# Autodesk Inventor assembly: Ensamble v2
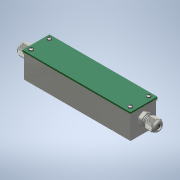
[picture p0: Inventor's stored thumbnail of the model, 180x180]
Saved by Autodesk Inventor 2021 (Build 250183000, 183)
## iProperties
Created: 2021-03-08
Part Number: Ensamble v2
Material: Generic
Document SubType Name: Assembly
Designer: Usuario
Author: Usuario
## Documents named in this file (8)
- C:\Users\Usuario\Desktop\INVENTOR\v 0.2\Ensamble v2.iam
- C:\Users\Usuario\Desktop\INVENTOR\v 0.2\base inferior.ipt
- C:\Users\Usuario\Desktop\INVENTOR\Componentes\PG7 Cable Gland.ipt
- C:\Users\Usuario\Desktop\INVENTOR\v 0.2\tapa.ipt
- C:\Users\Usuario\Desktop\INVENTOR\Componentes\Arduino\Arduino Nano R3 ATmega 328P.iam
- C:\Users\Usuario\Desktop\INVENTOR\Componentes\rs485.ipt
- C:\Users\Usuario\Desktop\INVENTOR\Componentes\SX1308_STEPUP_DCDC.ipt
- C:\Users\Usuario\Documents\Inventor\Content Center Files\R2021\en-US\BS EN ISO 7045 H\EN ISO 7045 - M3 x 10 - 4.8 - H(1).ipt
## Components (11 placed, 7 different names)
1. base inferior:1 — Insert:1, Insert:2, Mate:1, Flush:1, Mate:2, Mate:3, Mate:4
2. PG7 Cable Gland:1 — Insert:1
3. PG7 Cable Gland:2 — Insert:2
4. tapa:1 — Mate:1, Flush:1, Insert:3, Insert:4, Insert:5, Insert:6
5. Arduino Nano R3 ATmega 328P:1 [sub-assembly] — Mate:3
6. rs485:1 — Mate:4
7. SX1308_STEPUP_DCDC:1 — Mate:2
8. BS EN ISO 7045 H - Metric M3 x 10 - 4.8 - H:1 — Insert:4
9. BS EN ISO 7045 H - Metric M3 x 10 - 4.8 - H:2 — Insert:3
10. BS EN ISO 7045 H - Metric M3 x 10 - 4.8 - H:3 — Insert:6
11. BS EN ISO 7045 H - Metric M3 x 10 - 4.8 - H:4 — Insert:5
## Relationships (11: Insert 6, Mate 4, Flush 1)
- Insert:1: base inferior:1 ↔ PG7 Cable Gland:1
- Insert:2: base inferior:1 ↔ PG7 Cable Gland:2
- Mate:1: base inferior:1 ↔ tapa:1
- Flush:1: base inferior:1 ↔ tapa:1
- Mate:2: base inferior:1 ↔ SX1308_STEPUP_DCDC:1
- Mate:3: base inferior:1 ↔ Arduino Nano R3 ATmega 328P:1
- Mate:4: base inferior:1 ↔ rs485:1
- Insert:3: tapa:1 ↔ BS EN ISO 7045 H - Metric M3 x 10 - 4.8 - H:2
- Insert:4: tapa:1 ↔ BS EN ISO 7045 H - Metric M3 x 10 - 4.8 - H:1
- Insert:5: tapa:1 ↔ BS EN ISO 7045 H - Metric M3 x 10 - 4.8 - H:4
- Insert:6: tapa:1 ↔ BS EN ISO 7045 H - Metric M3 x 10 - 4.8 - H:3
